# Autodesk Inventor assembly: brideye_camera_realsense
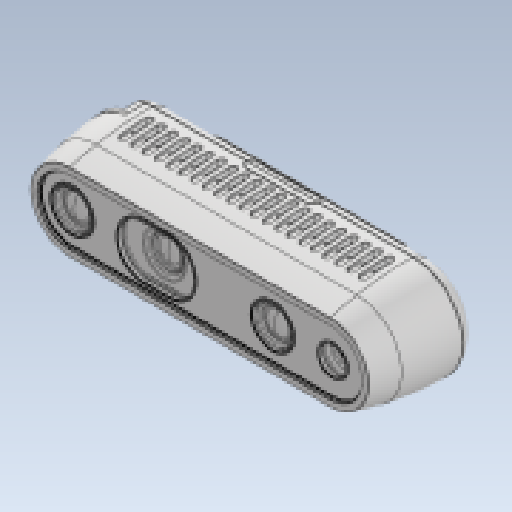
[picture p0: Inventor's stored thumbnail of the model, 512x512]
Saved by Autodesk Inventor 2024 (Build 280153000, 153)
## iProperties
Created: 2023-09-30
Part Number: brideye_camera_realsense
Document SubType Name: Assembly
Designer: michi
Author: michi
## Documents named in this file (3)
- C:\Users\michi\OneDrive - Kyoto University\lab\6_SHINOBI\FUHGA4\Design_Mechanism\05_birdeye\birdeye_wristUnit\realsense.iam
- C:\Users\michi\OneDrive - Kyoto University\lab\6_SHINOBI\FUHGA4\Design_Mechanism\00_devices\Camera-Stereo_RealSense\Intel_RealSense_Depth_Camera_D435.iam
- C:\Users\michi\OneDrive - Kyoto University\lab\6_SHINOBI\FUHGA4\Design_Mechanism\05_birdeye\birdeye_wristUnit\realsense_adapter.ipt
## Components (2 placed, 2 different names)
1. Intel_RealSense_Depth_Camera_D435:1 [sub-assembly] — 回転:1, 回転:2
2. realsense_adapter:1 — 回転:1, 回転:2
## Relationships (2: RevoluteJoint 2)
- 回転:1 [RevoluteJoint]: Intel_RealSense_Depth_Camera_D435:1 ↔ realsense_adapter:1
- 回転:2 [RevoluteJoint]: Intel_RealSense_Depth_Camera_D435:1 ↔ realsense_adapter:1
